# Autodesk Inventor assembly: gorne_ramie_wahacz_tylny
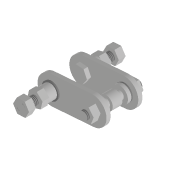
[picture p0: Inventor's stored thumbnail of the model, 180x180]
Saved by Autodesk Inventor 2020.3 (Build 243373000, 373)
## iProperties
Created: 2022-01-11
Part Number: gorne_ramie_wahacz_tylny
Document SubType Name: Assembly
Designer: patry
Author: patry
## Documents named in this file (9)
- C:\Users\patry\Desktop\Semestr 7\Inzynierka\Projekt inventor\Ariadna_inzynierka\Workspaces\Obszar roboczy\Obszar roboczy\Naped\Zawieszenie_v3\gorne_ramie_wahacz_tylny.iam
- C:\Users\patry\Desktop\Semestr 7\Inzynierka\Projekt inventor\Ariadna_inzynierka\Workspaces\Obszar roboczy\Obszar roboczy\Naped\Zawieszenie_v3\tuleja_TUF106040.ipt
- C:\Users\patry\Desktop\Semestr 7\Inzynierka\Projekt inventor\Ariadna_inzynierka\Workspaces\Obszar roboczy\Obszar roboczy\Naped\Sruby\M6_40_shaft.ipt
- C:\Users\patry\Desktop\Semestr 7\Inzynierka\Projekt inventor\Ariadna_inzynierka\Workspaces\Obszar roboczy\Obszar roboczy\Naped\Sruby\M6_nut_5mm.ipt
- C:\Users\patry\Desktop\Semestr 7\Inzynierka\Projekt inventor\Ariadna_inzynierka\Workspaces\Obszar roboczy\Obszar roboczy\Naped\Sruby\tuleja_M6_M10_7.ipt
- C:\Users\patry\Desktop\Semestr 7\Inzynierka\Projekt inventor\Ariadna_inzynierka\Workspaces\Obszar roboczy\Obszar roboczy\Naped\Sruby\M6_1,25_pad.ipt
- C:\Users\patry\Desktop\Semestr 7\Inzynierka\Projekt inventor\Ariadna_inzynierka\Workspaces\Obszar roboczy\Obszar roboczy\Naped\Sruby\tuleja_M6_M10_6.ipt
- C:\Users\patry\Desktop\Semestr 7\Inzynierka\Projekt inventor\Ariadna_inzynierka\Workspaces\Obszar roboczy\Obszar roboczy\Naped\Zawieszenie_v3\ramie_2_wahacza_tylnego.ipt
- C:\Users\patry\Desktop\Semestr 7\Inzynierka\Projekt inventor\Ariadna_inzynierka\Workspaces\Obszar roboczy\Obszar roboczy\Naped\Sruby\M6x25_plaski_leb.ipt
## Components (22 placed, 8 different names)
1. tuleja_TUF106040:1
2. tuleja_TUF106040:2
3. tuleja_TUF106040:3
4. tuleja_TUF106040:4
5. M6_40_shaft:1
6. M6_nut_5mm:1
7. M6_nut_5mm:2
8. tuleja_M6_M10_7:1
9. M6_1,25_pad:1
10. M6_1,25_pad:2
11. M6_1,25_pad:3
12. M6_1,25_pad:4
13. M6_nut_5mm:3
14. M6_nut_5mm:4
15. M6_nut_5mm:5
16. M6_nut_5mm:6
17. tuleja_M6_M10_6:1
18. tuleja_M6_M10_6:2
19. ramie_2_wahacza_tylnego:1
20. ramie_2_wahacza_tylnego:2
21. M6x25_plaski_leb:1
22. M6x25_plaski_leb:2
## Relationships (41: Mate 40, Flush 1)
- [Mate]: tuleja_TUF106040:1 ↔ tuleja_TUF106040:3
- [Mate]: tuleja_TUF106040:3 ↔ M6_40_shaft:1
- [Mate]: M6_40_shaft:1 ↔ M6_nut_5mm:1
- [Mate]: M6_40_shaft:1 ↔ M6_nut_5mm:2
- [Mate]: M6_40_shaft:1 ↔ tuleja_M6_M10_7:1
- [Mate]: M6_1,25_pad:1 ↔ M6_1,25_pad:2
- [Mate]: M6_1,25_pad:1 ↔ M6_1,25_pad:2
- [Mate]: M6_40_shaft:1 ↔ M6_1,25_pad:1
- [Mate]: M6_1,25_pad:3 ↔ M6_1,25_pad:4
- [Mate]: M6_1,25_pad:3 ↔ M6_1,25_pad:4
- [Mate]: M6_40_shaft:1 ↔ M6_1,25_pad:3
- [Mate]: tuleja_TUF106040:3 ↔ M6_1,25_pad:3
- [Mate] (60 mm): M6_nut_5mm:3 ↔ M6_nut_5mm:4
- [Mate]: M6_nut_5mm:3 ↔ M6_nut_5mm:4
- [Mate]: tuleja_TUF106040:1 ↔ M6_1,25_pad:2
- [Mate] (5 mm): M6_nut_5mm:4 ↔ M6_nut_5mm:5
- [Mate] (5 mm): M6_nut_5mm:3 ↔ M6_nut_5mm:6
- [Mate]: tuleja_TUF106040:4 ↔ tuleja_M6_M10_6:1
- [Mate]: tuleja_TUF106040:2 ↔ tuleja_M6_M10_6:2
- [Mate]: tuleja_TUF106040:1 ↔ ramie_2_wahacza_tylnego:1
- [Mate]: tuleja_TUF106040:1 ↔ ramie_2_wahacza_tylnego:1
- [Mate]: tuleja_TUF106040:2 ↔ ramie_2_wahacza_tylnego:1
- [Mate]: tuleja_TUF106040:2 ↔ ramie_2_wahacza_tylnego:1
- [Mate]: M6_nut_5mm:4 ↔ M6_nut_5mm:5
- [Mate] (5 mm): M6_nut_5mm:4 ↔ M6_nut_5mm:5
- [Mate]: M6_nut_5mm:5 ↔ tuleja_M6_M10_6:2
- [Mate]: tuleja_TUF106040:2 ↔ M6_nut_5mm:5
- [Mate]: tuleja_TUF106040:3 ↔ ramie_2_wahacza_tylnego:2
- [Mate]: tuleja_TUF106040:3 ↔ ramie_2_wahacza_tylnego:2
- [Mate]: tuleja_TUF106040:4 ↔ ramie_2_wahacza_tylnego:2
- [Mate]: tuleja_TUF106040:4 ↔ ramie_2_wahacza_tylnego:2
- [Mate]: tuleja_TUF106040:4 ↔ tuleja_M6_M10_6:1
- [Mate]: M6_nut_5mm:6 ↔ tuleja_M6_M10_6:1
- [Mate]: M6_nut_5mm:3 ↔ M6_nut_5mm:6
- [Mate]: M6_nut_5mm:6 ↔ M6x25_plaski_leb:2
- [Mate]: ramie_2_wahacza_tylnego:2 ↔ M6x25_plaski_leb:2
- [Mate]: tuleja_TUF106040:2 ↔ M6x25_plaski_leb:1
- [Mate]: ramie_2_wahacza_tylnego:1 ↔ M6x25_plaski_leb:1
- [Mate]: M6_nut_5mm:2 ↔ ramie_2_wahacza_tylnego:2
- [Mate]: M6_nut_5mm:1 ↔ ramie_2_wahacza_tylnego:1
- [Flush] (-2 mm): M6_40_shaft:1 ↔ M6_nut_5mm:1
## Named parameters: d178_d176 = 60 mm, d162_d154 = 0 mm, d163_d155 = 0 mm, d166_d154 = 0 mm, d167_d155 = 0 mm
